# Autodesk Inventor assembly: LR_00
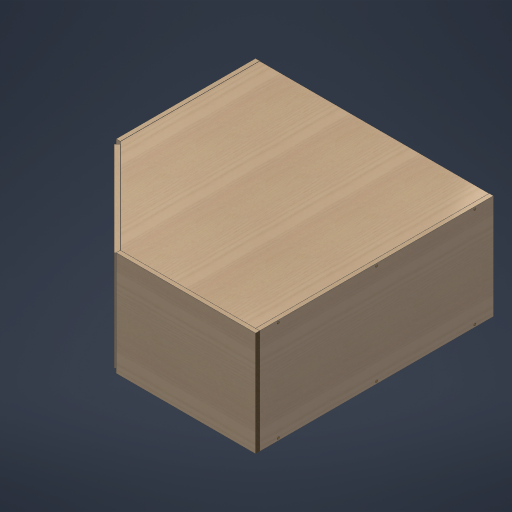
[picture p0: Inventor's stored thumbnail of the model, 512x512]
Saved by Autodesk Inventor 2024.3 (Build 283343000, 343)
## iProperties
Created: 2013-04-02
Part Number: LR_00
Document SubType Name: Assembly
Designer: User
Description: Entresol
Material Code: Item.FillWorkpiece.Material.Code
Author: User
## Documents named in this file (15)
- C:\W4INV 2024 Design\PROJECTS\Living Room\Entresol\LR_00.iam
- C:\W4INV 2024 Design\PROJECTS\Samples\Living Room\Entresol\LR_0000.ipt
- C:\W4INV 2024 Design\PROJECTS\Samples\Living Room\Entresol\LR_0003.ipt
- C:\W4INV 2024 Design\PROJECTS\Samples\Living Room\Entresol\LR_0004.ipt
- C:\W4INV 2024 Design\PROJECTS\Samples\Living Room\Entresol\LR_0006.ipt
- C:\W4INV 2024 Design\PROJECTS\Samples\Living Room\Entresol\LR_0001.ipt
- C:\W4INV 2024 Design\PROJECTS\Samples\Living Room\Entresol\LR_0002.ipt
- C:\W4INV 2024 Design\PROJECTS\Samples\Living Room\Entresol\LR_0005.ipt
- C:\W4INV 2024 Design\_LIBRARY\Fixed joints\Confirmat\CONFIRMAT\Confirmat L50 & Cap D10 NB T18 PB T 18.ipt
- C:\W4INV 2024 Design\_LIBRARY\Fixed joints\Minifix joint\MINIFIX D15 v2\Minifix D15 & Dowel L34 & Cap D15 PB T18 LH.ipt
- C:\W4INV 2024 Design\_LIBRARY\Fixed joints\Minifix joint\MINIFIX D15 v2\Minifix D15 & Dowel L34 & Cap D15 PB T18 RH.ipt
- C:\W4INV 2024 Design\_LIBRARY\Hinges\45 DEGREE HINGE\45 Degree Hinge with Wood Screws And Cup Fixing Wood Screws.iam
- C:\W4INV 2024 Design\LIBRARY\Fixed joints\Confirmat\CONFIRMAT.ipt
- C:\W4INV 2024 Design\LIBRARY\Fixed joints\Minifix joint\MINIFIX D15 v2.ipt
- C:\W4INV 2024 Design\LIBRARY\Hinges\45 DEGREE HINGE.iam
## Components (23 placed, 11 different names)
1. LR_0000-Right Side:1 — Flush:3, Flush:4, Mate:50, Mate:52, Mate:54, Mate:56
2. LR_0003-Left Side:1 — Flush:1, Flush:2, Mate:26, Mate:30, Mate:34, Mate:38, Flush:67, Mate:58, Flush:68, Mate:60
3. LR_0004-Back:1 — Mate:1, Flush:27, Mate:3, Flush:28, Mate:5, Flush:29, Mate:7, Flush:30, Mate:9, Flush:31, Mate:11, Flush:32
4. LR_0006-Top:1 — Mate:2, Mate:6, Mate:10, Flush:51, Flush:55, Flush:63, Flush:65
5. LR_0001-Bottom:1 — Mate:4, Mate:8, Mate:12, Flush:53, Flush:57, Flush:64, Flush:66
6. LR_0002-Door:1 — Flush:25, Flush:26
7. LR_0005-Back:1
8. Confirmat L50 & Cap D10 NB T18 PB T 18:2 — Mate:1, Mate:2, Flush:27
9. Confirmat L50 & Cap D10 NB T18 PB T 18:3 — Mate:3, Mate:4, Flush:28
10. Confirmat L50 & Cap D10 NB T18 PB T 18:4 — Mate:5, Mate:6, Flush:29
11. Confirmat L50 & Cap D10 NB T18 PB T 18:5 — Mate:7, Mate:8, Flush:30
12. Confirmat L50 & Cap D10 NB T18 PB T 18:6 — Mate:9, Mate:10, Flush:31
13. Confirmat L50 & Cap D10 NB T18 PB T 18:7 — Mate:11, Mate:12, Flush:32
14. Minifix D15 & Dowel L34 & Cap D15 PB T18 LH:1 — Mate:25, Flush:51, Mate:26
15. Minifix D15 & Dowel L34 & Cap D15 PB T18 RH:3 — Mate:29, Flush:53, Mate:30
16. Minifix D15 & Dowel L34 & Cap D15 PB T18 RH:5 — Mate:33, Flush:55, Mate:34
17. Minifix D15 & Dowel L34 & Cap D15 PB T18 LH:7 — Mate:37, Flush:57, Mate:38
18. Minifix D15 & Dowel L34 & Cap D15 PB T18 LH:13 — Mate:49, Flush:63, Mate:50
19. Minifix D15 & Dowel L34 & Cap D15 PB T18 RH:14 — Mate:51, Flush:64, Mate:52
20. Minifix D15 & Dowel L34 & Cap D15 PB T18 RH:15 — Mate:53, Flush:65, Mate:54
21. Minifix D15 & Dowel L34 & Cap D15 PB T18 LH:16 — Mate:55, Flush:66, Mate:56
22. 45 Degree Hinge with Wood Screws And Cup Fixing Wood Screws:2 [sub-assembly] — Mate:57, Flush:67, Mate:58
23. 45 Degree Hinge with Wood Screws And Cup Fixing Wood Screws:3 [sub-assembly] — Mate:59, Flush:68, Mate:60
## Relationships (54: Mate 32, Flush 22)
- Flush:1 (-80 mm): LR_0003-Left Side:1
- Flush:2 (-80 mm): LR_0003-Left Side:1
- Flush:3 (-80 mm): LR_0000-Right Side:1
- Flush:4 (-80 mm): LR_0000-Right Side:1
- Flush:25 (-50 mm): LR_0002-Door:1
- Flush:26 (-50 mm): LR_0002-Door:1
- Mate:1: LR_0004-Back:1 ↔ Confirmat L50 & Cap D10 NB T18 PB T 18:2
- Mate:2 (-9 mm): LR_0006-Top:1 ↔ Confirmat L50 & Cap D10 NB T18 PB T 18:2
- Flush:27: LR_0004-Back:1 ↔ Confirmat L50 & Cap D10 NB T18 PB T 18:2
- Mate:3: LR_0004-Back:1 ↔ Confirmat L50 & Cap D10 NB T18 PB T 18:3
- Mate:4 (-9 mm): LR_0001-Bottom:1 ↔ Confirmat L50 & Cap D10 NB T18 PB T 18:3
- Flush:28: LR_0004-Back:1 ↔ Confirmat L50 & Cap D10 NB T18 PB T 18:3
- Mate:5: LR_0004-Back:1 ↔ Confirmat L50 & Cap D10 NB T18 PB T 18:4
- Mate:6 (-9 mm): LR_0006-Top:1 ↔ Confirmat L50 & Cap D10 NB T18 PB T 18:4
- Flush:29: LR_0004-Back:1 ↔ Confirmat L50 & Cap D10 NB T18 PB T 18:4
- Mate:7: LR_0004-Back:1 ↔ Confirmat L50 & Cap D10 NB T18 PB T 18:5
- Mate:8 (-9 mm): LR_0001-Bottom:1 ↔ Confirmat L50 & Cap D10 NB T18 PB T 18:5
- Flush:30: LR_0004-Back:1 ↔ Confirmat L50 & Cap D10 NB T18 PB T 18:5
- Mate:9: LR_0004-Back:1 ↔ Confirmat L50 & Cap D10 NB T18 PB T 18:6
- Mate:10 (-9 mm): LR_0006-Top:1 ↔ Confirmat L50 & Cap D10 NB T18 PB T 18:6
- Flush:31: LR_0004-Back:1 ↔ Confirmat L50 & Cap D10 NB T18 PB T 18:6
- Mate:11: LR_0004-Back:1 ↔ Confirmat L50 & Cap D10 NB T18 PB T 18:7
- Mate:12 (-9 mm): LR_0001-Bottom:1 ↔ Confirmat L50 & Cap D10 NB T18 PB T 18:7
- Flush:32: LR_0004-Back:1 ↔ Confirmat L50 & Cap D10 NB T18 PB T 18:7
- Mate:25: Minifix D15 & Dowel L34 & Cap D15 PB T18 LH:1
- Flush:51 (18 mm): LR_0006-Top:1 ↔ Minifix D15 & Dowel L34 & Cap D15 PB T18 LH:1
- Mate:26: LR_0003-Left Side:1 ↔ Minifix D15 & Dowel L34 & Cap D15 PB T18 LH:1
- Mate:29: Minifix D15 & Dowel L34 & Cap D15 PB T18 RH:3
- Flush:53 (18 mm): LR_0001-Bottom:1 ↔ Minifix D15 & Dowel L34 & Cap D15 PB T18 RH:3
- Mate:30: LR_0003-Left Side:1 ↔ Minifix D15 & Dowel L34 & Cap D15 PB T18 RH:3
- Mate:33: Minifix D15 & Dowel L34 & Cap D15 PB T18 RH:5
- Flush:55 (18 mm): LR_0006-Top:1 ↔ Minifix D15 & Dowel L34 & Cap D15 PB T18 RH:5
- Mate:34: LR_0003-Left Side:1 ↔ Minifix D15 & Dowel L34 & Cap D15 PB T18 RH:5
- Mate:37: Minifix D15 & Dowel L34 & Cap D15 PB T18 LH:7
- Flush:57 (18 mm): LR_0001-Bottom:1 ↔ Minifix D15 & Dowel L34 & Cap D15 PB T18 LH:7
- Mate:38: LR_0003-Left Side:1 ↔ Minifix D15 & Dowel L34 & Cap D15 PB T18 LH:7
- Mate:49: Minifix D15 & Dowel L34 & Cap D15 PB T18 LH:13
- Flush:63 (18 mm): LR_0006-Top:1 ↔ Minifix D15 & Dowel L34 & Cap D15 PB T18 LH:13
- Mate:50: LR_0000-Right Side:1 ↔ Minifix D15 & Dowel L34 & Cap D15 PB T18 LH:13
- Mate:51: Minifix D15 & Dowel L34 & Cap D15 PB T18 RH:14
- Flush:64 (18 mm): LR_0001-Bottom:1 ↔ Minifix D15 & Dowel L34 & Cap D15 PB T18 RH:14
- Mate:52: LR_0000-Right Side:1 ↔ Minifix D15 & Dowel L34 & Cap D15 PB T18 RH:14
- Mate:53: Minifix D15 & Dowel L34 & Cap D15 PB T18 RH:15
- Flush:65 (18 mm): LR_0006-Top:1 ↔ Minifix D15 & Dowel L34 & Cap D15 PB T18 RH:15
- Mate:54: LR_0000-Right Side:1 ↔ Minifix D15 & Dowel L34 & Cap D15 PB T18 RH:15
- Mate:55: Minifix D15 & Dowel L34 & Cap D15 PB T18 LH:16
- Flush:66 (18 mm): LR_0001-Bottom:1 ↔ Minifix D15 & Dowel L34 & Cap D15 PB T18 LH:16
- Mate:56: LR_0000-Right Side:1 ↔ Minifix D15 & Dowel L34 & Cap D15 PB T18 LH:16
- Mate:57: 45 Degree Hinge with Wood Screws And Cup Fixing Wood Screws:2
- Flush:67 (37 mm): LR_0003-Left Side:1 ↔ 45 Degree Hinge with Wood Screws And Cup Fixing Wood Screws:2
- Mate:58: LR_0003-Left Side:1 ↔ 45 Degree Hinge with Wood Screws And Cup Fixing Wood Screws:2
- Mate:59: 45 Degree Hinge with Wood Screws And Cup Fixing Wood Screws:3
- Flush:68 (37 mm): LR_0003-Left Side:1 ↔ 45 Degree Hinge with Wood Screws And Cup Fixing Wood Screws:3
- Mate:60: LR_0003-Left Side:1 ↔ 45 Degree Hinge with Wood Screws And Cup Fixing Wood Screws:3
